# Autodesk Inventor assembly: Tarraxa
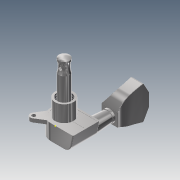
[picture p0: Inventor's stored thumbnail of the model, 180x180]
Saved by Autodesk Inventor 2016 (Build 200138000, 138)
## iProperties
Created: 2018-12-06
Part Number: Tarraxa
Document SubType Name: Assembly
Designer: dqm_r
Author: dqm_r
## Documents named in this file (4)
- C:\Users\Pedro\Google Drive\Projeto CAD Eng Mecânica\Tarraxa.iam
- C:\Users\Pedro\Google Drive\Projeto CAD Eng Mecânica\Peça 7.ipt
- C:\Users\Pedro\Google Drive\Projeto CAD Eng Mecânica\Cabeça da tarraxa.ipt
- C:\Users\Pedro\Google Drive\Projeto CAD Eng Mecânica\Parafuso menor Tarraxa.ipt
## Components (3 placed, 3 different names)
1. Peça 7:1 — Mate:1, Rotational:1
2. Cabeça da tarraxa:1 — Mate:1, Rotational:1, Insert:1
3. Parafuso menor Tarraxa:1 — Insert:1
## Relationships (3: Mate 1, RevoluteJoint 1, Insert 1)
- Mate:1: Peça 7:1 ↔ Cabeça da tarraxa:1
- Rotational:1 [RevoluteJoint]: Peça 7:1 ↔ Cabeça da tarraxa:1
- Insert:1: Cabeça da tarraxa:1 ↔ Parafuso menor Tarraxa:1
